# Autodesk Inventor assembly: base_assembly
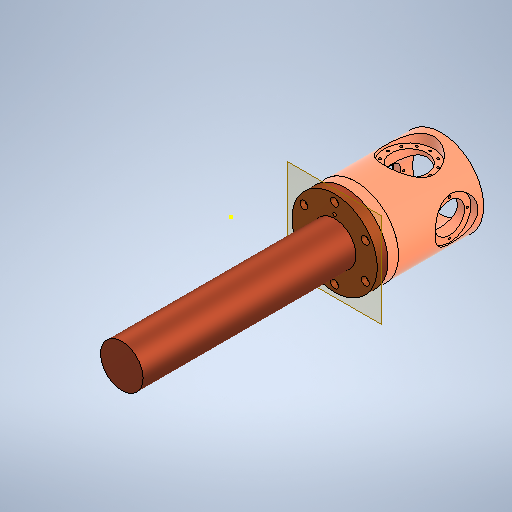
[picture p0: Inventor's stored thumbnail of the model, 512x512]
Saved by Autodesk Inventor 2026.1 (Build 301233000, 233)
## iProperties
Created: 2018-08-22
Part Number: base_assembly
Document SubType Name: Assembly
Designer: Q
Mass: 15991.1 g
Surface Area: 2076.34 cm^2
Volume: 1788.71 cm^3
Density: 8.94 g/cm^3
Author: Q
## Documents named in this file (9)
- C:\Users\user\Desktop\setup_inventor_2025\base\base_assembly.iam
- C:\Users\user\Desktop\setup_inventor_2025\base\base_becher.ipt
- C:\Users\user\Desktop\setup_inventor_2025\base\base_becherboden.ipt
- C:\Users\user\Desktop\setup_inventor_2025\base\base_connector.ipt
- C:\Users\user\Desktop\setup_inventor_2025\base\base_stange.ipt
- N:\intern\Kaufmann-Group\Projects\setup\inventor\base\base_becher.ipt
- N:\intern\Kaufmann-Group\Projects\setup\inventor\base\base_becherboden.ipt
- N:\intern\Kaufmann-Group\Projects\setup\inventor\base\base_connector.ipt
- N:\intern\Kaufmann-Group\Projects\setup\inventor\base\base_stange.ipt
## Components (4 placed, 4 different names)
1. base_becher:1 — Flush:1
2. base_becherboden:1 — Flush:1, Flush:2, Flush:3
3. base_connector:1 — Flush:2, Flush:3, Flush:4
4. base_stange:1 — Flush:4
## Relationships (4: Flush 4)
- Flush:1: base_becher:1 ↔ base_becherboden:1
- Flush:2: base_becherboden:1 ↔ base_connector:1
- Flush:3: base_becherboden:1 ↔ base_connector:1
- Flush:4: base_connector:1 ↔ base_stange:1
